# Autodesk Inventor assembly: INTEGRATED_SIDE_FRAME_007B_ASM
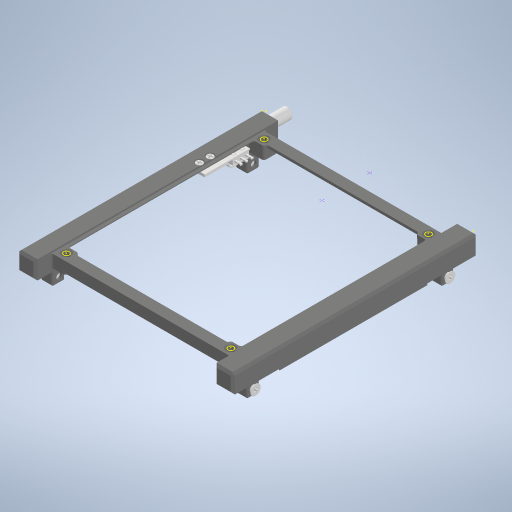
[picture p0: Inventor's stored thumbnail of the model, 512x512]
Saved by Autodesk Inventor 2023 (Build 270158000, 158)
## iProperties
Created: 2011-03-02
Part Number: INTEGRATED_SIDE_FRAME_007B_ASM
Description: NOT SPECIFIED
Document SubType Name: Assembly
Designer: maylo
Author: maylo
Revision Number: LAST_VERSION
## Documents named in this file (12)
- E:\Dropbox\AMSAT\Cube Sat Frame Info\ISIS\INTEGRATED_SIDE_FRAME_007B_ASM.iam
- E:\Dropbox\AMSAT\Cube Sat Frame Info\ISIS\KILL_SWITCH_AV46J_ASM.iam
- E:\Dropbox\AMSAT\Cube Sat Frame Info\ISIS\SCREW_M2_5X6.ipt
- E:\Dropbox\AMSAT\Cube Sat Frame Info\ISIS\BRACKET_KS_007B.ipt
- E:\Dropbox\AMSAT\Cube Sat Frame Info\ISIS\BRACKET_KS_007A.ipt
- E:\Dropbox\AMSAT\Cube Sat Frame Info\ISIS\BUSJE_001.ipt
- E:\Dropbox\AMSAT\Cube Sat Frame Info\ISIS\KILL_SWITCH_LEVER.ipt
- E:\Dropbox\AMSAT\Cube Sat Frame Info\ISIS\KILL_SWITCH_SWITCH.ipt
- E:\Dropbox\AMSAT\Cube Sat Frame Info\ISIS\SPRING_02.ipt
- E:\Dropbox\AMSAT\Cube Sat Frame Info\ISIS\KILL_SWITCH_PIN.ipt
- E:\Dropbox\AMSAT\Cube Sat Frame Info\ISIS\KS_MECH_SCREWS_ASM.iam
- E:\Dropbox\AMSAT\Cube Sat Frame Info\ISIS\SIDE_FRAME_007.ipt
## Components (14 placed, 14 different names)
1. KILL_SWITCH_AV46J_ASM_2 [sub-assembly]
2. SCREW_M2_5X6_3
3. SCREW_M2_5X6_4
4. BRACKET_KS_007B_5
5. BRACKET_KS_007A_6
6. SCREW_M2_5X6_7
7. BUSJE_001_8
8. KILL_SWITCH_LEVER_9
9. KILL_SWITCH_SWITCH_10
10. SPRING_02_11
11. SCREW_M2_5X6_12
12. KILL_SWITCH_PIN_13
13. KS_MECH_SCREWS_ASM_20 [sub-assembly]
14. SIDE_FRAME_007_21 — Mate:1, Angle:1
## Relationships (2: Mate 1, Angle 1)
- Mate:1: SIDE_FRAME_007_21
- Angle:1 (0 deg): SIDE_FRAME_007_21
